# Autodesk Inventor assembly: Growroom Assembly
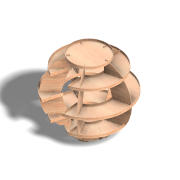
[picture p0: Inventor's stored thumbnail of the model, 180x180]
Saved by Autodesk Inventor 2021 (Build 250183000, 183)
## iProperties
Created: 2020-03-07
Part Number: Growroom Assembly
Document SubType Name: Assembly
Designer: Daniel Wikman
Author: Daniel Wikman
## Documents named in this file (23)
- C:\Users\Dan Wikman\OneDrive\University Life\2020, Semester 1\METR4900 Honours Thesis\Prototype CAD\Growroom Assembly.iam
- C:\Users\Dan Wikman\OneDrive\University Life\2020, Semester 1\METR4900 Honours Thesis\Prototype CAD\Base - A.ipt
- C:\Users\Dan Wikman\OneDrive\University Life\2020, Semester 1\METR4900 Honours Thesis\Prototype CAD\Support A.ipt
- C:\Users\Dan Wikman\OneDrive\University Life\2020, Semester 1\METR4900 Honours Thesis\Prototype CAD\Support A1.ipt
- C:\Users\Dan Wikman\OneDrive\University Life\2020, Semester 1\METR4900 Honours Thesis\Prototype CAD\Support A Cross.ipt
- C:\Users\Dan Wikman\OneDrive\University Life\2020, Semester 1\METR4900 Honours Thesis\Prototype CAD\Support A Cross Dual1.ipt
- C:\Users\Dan Wikman\OneDrive\University Life\2020, Semester 1\METR4900 Honours Thesis\Prototype CAD\Support A Cross Dual2.ipt
- C:\Users\Dan Wikman\OneDrive\University Life\2020, Semester 1\METR4900 Honours Thesis\Prototype CAD\Ring B Assembly.iam
- C:\Users\Dan Wikman\OneDrive\University Life\2020, Semester 1\METR4900 Honours Thesis\Prototype CAD\Wedge.ipt
- C:\Users\Dan Wikman\OneDrive\University Life\2020, Semester 1\METR4900 Honours Thesis\Prototype CAD\Feet.ipt
- C:\Users\Dan Wikman\OneDrive\University Life\2020, Semester 1\METR4900 Honours Thesis\Prototype CAD\Support B.ipt
- C:\Users\Dan Wikman\OneDrive\University Life\2020, Semester 1\METR4900 Honours Thesis\Prototype CAD\Ring C Assembly.iam
- C:\Users\Dan Wikman\OneDrive\University Life\2020, Semester 1\METR4900 Honours Thesis\Prototype CAD\Support C.ipt
- C:\Users\Dan Wikman\OneDrive\University Life\2020, Semester 1\METR4900 Honours Thesis\Prototype CAD\Ring D Assembly.iam
- C:\Users\Dan Wikman\OneDrive\University Life\2020, Semester 1\METR4900 Honours Thesis\Prototype CAD\Support D.ipt
- C:\Users\Dan Wikman\OneDrive\University Life\2020, Semester 1\METR4900 Honours Thesis\Prototype CAD\Roof - G.ipt
- C:\Users\Dan Wikman\OneDrive\University Life\2020, Semester 1\METR4900 Honours Thesis\Prototype CAD\Banding Roof.ipt
- C:\Users\Dan Wikman\OneDrive\University Life\2020, Semester 1\METR4900 Honours Thesis\Prototype CAD\Banding Base.ipt
- C:\Users\Dan Wikman\OneDrive\University Life\2020, Semester 1\METR4900 Honours Thesis\Prototype CAD\Banding Level A-C Outer.ipt
- C:\Users\Dan Wikman\OneDrive\University Life\2020, Semester 1\METR4900 Honours Thesis\Prototype CAD\Banding Ends.ipt
- C:\Users\Dan Wikman\OneDrive\University Life\2020, Semester 1\METR4900 Honours Thesis\Prototype CAD\Banding Level A-C Inner.ipt
- C:\Users\Dan Wikman\OneDrive\University Life\2020, Semester 1\METR4900 Honours Thesis\Prototype CAD\Banding Mid Level Outer.ipt
- C:\Users\Dan Wikman\OneDrive\University Life\2020, Semester 1\METR4900 Honours Thesis\Prototype CAD\Banding Mid Level Inner.ipt
## Components (81 placed, 22 different names)
1. Base - A:1 — Mate:1, Mate:2, Mate:4, Mate:5, Mate:7, Mate:8, Mate:9, Mate:10, Mate:11, Mate:12, Mate:13, Mate:14, Mate:15, Mate:16, Mate:17, Mate:18, Mate:19, Mate:21, Mate:22, Mate:24, Mate:25, Mate:27, Mate:28, Mate:29, Mate:31, Mate:32, Mate:33, Mate:34, Mate:36, Mate:37, Mate:39, Mate:40, Mate:42, Mate:43, Mate:45, Mate:46, Mate:48, Mate:49, Mate:51, Mate:52, Mate:54, Mate:55, Mate:69, Mate:75, Mate:89, Mate:137, Mate:165
2. Support A:4 — Mate:1, Mate:2, Mate:11, Mate:35
3. Support A:5 — Mate:4, Mate:5, Mate:10, Mate:38, Mate:115, Flush:3, Flush:5, Mate:136
4. Support A:6 — Mate:15, Mate:16, Mate:17, Mate:41, Mate:50
5. Support A:7 — Mate:12, Mate:13, Mate:14, Mate:44, Mate:53, Mate:70, Mate:71, Mate:76, Mate:77, Flush:2, Mate:106, Mate:114, Mate:117
6. Support A:8 — Mate:7, Mate:8, Mate:9, Mate:47, Mate:56
7. Support A1:1 — Mate:24, Mate:25, Mate:69
8. Support A1:2 — Mate:21, Mate:22, Mate:31
9. Support A1:3 — Mate:27, Mate:28, Mate:29
10. Support A1:4 — Mate:18, Mate:19, Mate:32
11. Support A Cross:1 — Mate:33, Mate:34, Mate:35
12. Support A Cross:2 — Mate:36, Mate:37, Mate:38
13. Support A Cross Dual1:1 — Mate:42, Mate:43, Mate:44
14. Support A Cross Dual1:2 — Mate:39, Mate:40, Mate:41
15. Support A Cross Dual1:3 — Mate:45, Mate:46, Mate:47
16. Support A Cross Dual2:1 — Mate:51, Mate:52, Mate:53
17. Support A Cross Dual2:2 — Mate:54, Mate:55, Mate:56
18. Support A Cross Dual2:3 — Mate:48, Mate:49, Mate:50
19. Ring B Assembly:1 [sub-assembly] — Mate:70, Mate:71, Mate:116, Mate:117, Mate:139, Flush:6, Mate:140, Mate:150, Mate:151, Mate:152
20. Ring C Assembly:1 [sub-assembly] — Mate:118, Mate:119, Mate:120, Mate:123, Mate:124, Mate:125, Mate:156, Mate:157, Mate:158, Mate:159, Mate:160, Mate:162
21. Ring D Assembly:1 [sub-assembly] — Mate:126, Mate:128, Mate:129, Mate:130, Mate:146, Flush:10, Flush:12, Mate:148, Mate:154
22. Roof - G:1 — Mate:131, Mate:132, Mate:133, Mate:134, Mate:135
23. Banding Roof:1 — Mate:134, Mate:135
24. Banding Base:1 — Flush:5, Mate:136, Mate:137
25. Banding Level A-C Outer:1 — Mate:138, Mate:139, Flush:6, Flush:7, Mate:141, Mate:153, Flush:15
26. Banding Ends:2 — Mate:140, Flush:7, Mate:141
27. Banding Level A-C Inner:1 — Mate:150, Mate:151
28. Banding Level A-C Outer:2 — Mate:146, Flush:10, Flush:11, Mate:147, Flush:14, Mate:149, Mate:155, Flush:16
29. Banding Level A-C Inner:2 — Mate:147, Flush:12, Flush:13
30. Banding Ends:3 — Mate:148, Flush:14, Mate:149
31. Banding Ends:4 — Mate:154, Mate:155, Flush:16
32. Banding Ends:5 — Mate:152, Mate:153, Flush:15
33. Banding Mid Level Outer:1 — Mate:156, Flush:17, Mate:157, Flush:18, Flush:19, Mate:161, Flush:20, Mate:163
34. Banding Mid Level Inner:1 — Mate:158, Mate:159, Flush:18
35. Banding Ends:6 — Mate:160, Flush:19, Mate:161
36. Banding Ends:7 — Mate:162, Flush:20, Mate:163
37. Feet:2 — Mate:81, Mate:82, Mate:83, Mate:106, Mate:164, Flush:21, Flush:22
38. Feet:3 — Mate:81, Mate:82, Mate:83, Mate:84, Mate:85, Mate:86
39. Feet:4 — Mate:84, Mate:85, Mate:86, Mate:89, Mate:95, Mate:114
40. Wedge:2 — Mate:73, Mate:74, Mate:77, Flush:2
41. Wedge:1 — Mate:73, Mate:74, Mate:75, Mate:76, Mate:95
42. Feet:8
43. Feet:9
44. Feet:10
45. Wedge:5
46. Wedge:6
47. Feet:11
48. Feet:12
49. Feet:13
50. Wedge:7
51. Wedge:8
52. Feet:14
53. Feet:15
54. Feet:16
55. Wedge:9
56. Wedge:10
57. Feet:17
58. Feet:18
59. Feet:19
60. Wedge:11
61. Wedge:12
62. Support B:1 — Mate:115, Mate:116, Flush:3, Mate:138
63. Support B:2
64. Support B:3
65. Support B:4 — Mate:118, Mate:119, Mate:120
66. Support B:5
67. Support C:1 — Mate:123, Mate:124, Mate:125, Mate:126, Mate:128, Flush:4
68. Support C:2
69. Support C:3 — Flush:17
70. Support C:4
71. Support C:5
72. Support D:1 — Mate:129, Flush:4, Mate:130, Mate:131, Mate:132, Mate:133
73. Support D:2
74. Support D:3 — Flush:11, Flush:13
75. Support D:4
76. Support D:5
77. Feet:20 — Mate:164, Flush:21, Flush:22
78. Feet:21
79. Feet:22
80. Feet:23
81. Feet:24
## Component patterns: (5 elements, first: Feet:2 + Feet:3 + Feet:4 + Wedge:2 + Wedge:1), (5 elements, first: Support B:1), (5 elements, first: Support C:1), (5 elements, first: Support D:1), (5 elements, first: Feet:20)
## Relationships (131: Mate 112, Flush 19)
- Mate:1: Base - A:1 ↔ Support A:4
- Mate:2 (0.25 mm): Base - A:1 ↔ Support A:4
- Mate:4: Base - A:1 ↔ Support A:5
- Mate:5 (0.25 mm): Base - A:1 ↔ Support A:5
- Mate:7: Base - A:1 ↔ Support A:8
- Mate:8 (0.25 mm): Base - A:1 ↔ Support A:8
- Mate:9 (1.3333 mm): Base - A:1 ↔ Support A:8
- Mate:10 (1.3333 mm): Base - A:1 ↔ Support A:5
- Mate:11 (1.3333 mm): Base - A:1 ↔ Support A:4
- Mate:12: Base - A:1 ↔ Support A:7
- Mate:13 (0.25 mm): Base - A:1 ↔ Support A:7
- Mate:14 (1.3333 mm): Base - A:1 ↔ Support A:7
- Mate:15: Base - A:1 ↔ Support A:6
- Mate:16 (0.25 mm): Base - A:1 ↔ Support A:6
- Mate:17 (1.3333 mm): Base - A:1 ↔ Support A:6
- Mate:18: Base - A:1 ↔ Support A1:4
- Mate:19 (0.25 mm): Base - A:1 ↔ Support A1:4
- Mate:21: Base - A:1 ↔ Support A1:2
- Mate:22 (0.25 mm): Base - A:1 ↔ Support A1:2
- Mate:24: Base - A:1 ↔ Support A1:1
- Mate:25 (0.25 mm): Base - A:1 ↔ Support A1:1
- Mate:27: Base - A:1 ↔ Support A1:3
- Mate:28 (0.25 mm): Base - A:1 ↔ Support A1:3
- Mate:29 (1.3333 mm): Base - A:1 ↔ Support A1:3
- Mate:31 (1.3333 mm): Base - A:1 ↔ Support A1:2
- Mate:32 (1.3333 mm): Base - A:1 ↔ Support A1:4
- Mate:33: Base - A:1 ↔ Support A Cross:1
- Mate:34 (0.25 mm): Base - A:1 ↔ Support A Cross:1
- Mate:35: Support A:4 ↔ Support A Cross:1
- Mate:36: Base - A:1 ↔ Support A Cross:2
- Mate:37 (0.25 mm): Base - A:1 ↔ Support A Cross:2
- Mate:38: Support A:5 ↔ Support A Cross:2
- Mate:39: Base - A:1 ↔ Support A Cross Dual1:2
- Mate:40 (0.25 mm): Base - A:1 ↔ Support A Cross Dual1:2
- Mate:41: Support A:6 ↔ Support A Cross Dual1:2
- Mate:42: Base - A:1 ↔ Support A Cross Dual1:1
- Mate:43 (0.25 mm): Base - A:1 ↔ Support A Cross Dual1:1
- Mate:44: Support A:7 ↔ Support A Cross Dual1:1
- Mate:45: Base - A:1 ↔ Support A Cross Dual1:3
- Mate:46 (0.25 mm): Base - A:1 ↔ Support A Cross Dual1:3
- Mate:47: Support A:8 ↔ Support A Cross Dual1:3
- Mate:48: Base - A:1 ↔ Support A Cross Dual2:3
- Mate:49 (0.25 mm): Base - A:1 ↔ Support A Cross Dual2:3
- Mate:50: Support A:6 ↔ Support A Cross Dual2:3
- Mate:51: Base - A:1 ↔ Support A Cross Dual2:1
- Mate:52 (0.25 mm): Base - A:1 ↔ Support A Cross Dual2:1
- Mate:53: Support A:7 ↔ Support A Cross Dual2:1
- Mate:54: Base - A:1 ↔ Support A Cross Dual2:2
- Mate:55 (0.25 mm): Base - A:1 ↔ Support A Cross Dual2:2
- Mate:56: Support A:8 ↔ Support A Cross Dual2:2
- Mate:69 (1.3333 mm): Base - A:1 ↔ Support A1:1
- Mate:70: Support A:7 ↔ Ring B Assembly:1
- Mate:71 (0.25 mm): Support A:7 ↔ Ring B Assembly:1
- Mate:73: Wedge:2 ↔ Wedge:1
- Mate:74: Wedge:2 ↔ Wedge:1
- Mate:75: Base - A:1 ↔ Wedge:1
- Mate:76 (0.25 mm): Support A:7 ↔ Wedge:1
- Mate:77: Support A:7 ↔ Wedge:2
- Mate:81: Feet:2 ↔ Feet:3
- Mate:82: Feet:2 ↔ Feet:3
- Mate:83: Feet:2 ↔ Feet:3
- Mate:84: Feet:3 ↔ Feet:4
- Mate:85: Feet:3 ↔ Feet:4
- Mate:86: Feet:3 ↔ Feet:4
- Mate:89: Base - A:1 ↔ Feet:4
- Mate:95 (0.25 mm): Feet:4 ↔ Wedge:1
- Flush:2 (-21.75 mm): Support A:7 ↔ Wedge:2
- Mate:106 (0.25 mm): Support A:7 ↔ Feet:2
- Mate:114 (0.25 mm): Support A:7 ↔ Feet:4
- Mate:115 (7.473 mm): Support A:5 ↔ Support B:1
- Mate:116: Ring B Assembly:1 ↔ Support B:1
- Flush:3: Support A:5 ↔ Support B:1
- Mate:117 (7.855 mm): Support A:7 ↔ Ring B Assembly:1
- Mate:118 (0.25 mm): Ring C Assembly:1 ↔ Support B:4
- Mate:119: Ring C Assembly:1 ↔ Support B:4
- Mate:120 (8.1885 mm): Ring C Assembly:1 ↔ Support B:4
- Mate:123: Ring C Assembly:1 ↔ Support C:1
- Mate:124: Ring C Assembly:1 ↔ Support C:1
- Mate:125 (0.25 mm): Ring C Assembly:1 ↔ Support C:1
- Mate:126 (0.25 mm): Ring D Assembly:1 ↔ Support C:1
- Mate:128 (7.855 mm): Ring D Assembly:1 ↔ Support C:1
- Mate:129: Ring D Assembly:1 ↔ Support D:1
- Flush:4: Support C:1 ↔ Support D:1
- Mate:130 (0.25 mm): Ring D Assembly:1 ↔ Support D:1
- Mate:131: Roof - G:1 ↔ Support D:1
- Mate:132 (0.25 mm): Roof - G:1 ↔ Support D:1
- Mate:133 (1.3333 mm): Roof - G:1 ↔ Support D:1
- Mate:134: Roof - G:1 ↔ Banding Roof:1
- Mate:135: Roof - G:1 ↔ Banding Roof:1
- Flush:5: Support A:5 ↔ Banding Base:1
- Mate:136: Support A:5 ↔ Banding Base:1
- Mate:137: Base - A:1 ↔ Banding Base:1
- Mate:138: Banding Level A-C Outer:1 ↔ Support B:1
- Mate:139: Ring B Assembly:1 ↔ Banding Level A-C Outer:1
- Flush:6: Ring B Assembly:1 ↔ Banding Level A-C Outer:1
- Mate:140: Ring B Assembly:1 ↔ Banding Ends:2
- Flush:7: Banding Level A-C Outer:1 ↔ Banding Ends:2
- Mate:141: Banding Level A-C Outer:1 ↔ Banding Ends:2
- Mate:146: Ring D Assembly:1 ↔ Banding Level A-C Outer:2
- Flush:10: Ring D Assembly:1 ↔ Banding Level A-C Outer:2
- Flush:11: Banding Level A-C Outer:2 ↔ Support D:3
- Mate:147: Banding Level A-C Outer:2 ↔ Banding Level A-C Inner:2
- Flush:12: Ring D Assembly:1 ↔ Banding Level A-C Inner:2
- Flush:13: Banding Level A-C Inner:2 ↔ Support D:3
- Mate:148: Ring D Assembly:1 ↔ Banding Ends:3
- Flush:14: Banding Level A-C Outer:2 ↔ Banding Ends:3
- Mate:149: Banding Level A-C Outer:2 ↔ Banding Ends:3
- Mate:150: Ring B Assembly:1 ↔ Banding Level A-C Inner:1
- Mate:151: Ring B Assembly:1 ↔ Banding Level A-C Inner:1
- Mate:152: Ring B Assembly:1 ↔ Banding Ends:5
- Mate:153: Banding Level A-C Outer:1 ↔ Banding Ends:5
- Flush:15: Banding Level A-C Outer:1 ↔ Banding Ends:5
- Mate:154: Ring D Assembly:1 ↔ Banding Ends:4
- Mate:155: Banding Level A-C Outer:2 ↔ Banding Ends:4
- Flush:16: Banding Level A-C Outer:2 ↔ Banding Ends:4
- Mate:156: Ring C Assembly:1 ↔ Banding Mid Level Outer:1
- Flush:17: Banding Mid Level Outer:1 ↔ Support C:3
- Mate:157: Ring C Assembly:1 ↔ Banding Mid Level Outer:1
- Mate:158: Ring C Assembly:1 ↔ Banding Mid Level Inner:1
- Mate:159: Ring C Assembly:1 ↔ Banding Mid Level Inner:1
- Flush:18: Banding Mid Level Outer:1 ↔ Banding Mid Level Inner:1
- Mate:160: Ring C Assembly:1 ↔ Banding Ends:6
- Flush:19: Banding Mid Level Outer:1 ↔ Banding Ends:6
- Mate:161: Banding Mid Level Outer:1 ↔ Banding Ends:6
- Mate:162: Ring C Assembly:1 ↔ Banding Ends:7
- Flush:20: Banding Mid Level Outer:1 ↔ Banding Ends:7
- Mate:163: Banding Mid Level Outer:1 ↔ Banding Ends:7
- Mate:164: Feet:2 ↔ Feet:20
- Flush:21: Feet:2 ↔ Feet:20
- Flush:22: Feet:2 ↔ Feet:20
- Mate:165: Base - A:1
